# Autodesk Inventor assembly: Robot Assembly
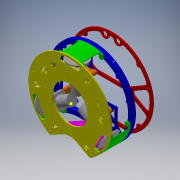
[picture p0: Inventor's stored thumbnail of the model, 180x180]
Saved by Autodesk Inventor 2018 (Build 220112000, 112)
## iProperties
Created: 2018-06-13
Part Number: Robot Assembly
Document SubType Name: Assembly
Designer: matth
Author: matth
## Documents named in this file (8)
- C:\Users\matth\Dropbox\M&A\Robotics-2018\Design and Hardware\Joinmax Parts\Robot Assembly.iam
- C:\Users\matth\Dropbox\M&A\Robotics-2018\Design and Hardware\Joinmax Parts\Base Plate.ipt
- C:\Users\matth\Dropbox\M&A\Robotics-2018\Design and Hardware\Joinmax Parts\Wheel Guard.ipt
- C:\Users\matth\Dropbox\M&A\Robotics-2018\Design and Hardware\Joinmax Parts\Joinmax.ipt
- C:\Users\matth\Dropbox\M&A\Robotics-2018\Design and Hardware\Joinmax Parts\Motor Standoff.ipt
- C:\Users\matth\Dropbox\M&A\Robotics-2018\Design and Hardware\Joinmax Parts\TSSP Ring.ipt
- C:\Users\matth\Dropbox\M&A\Robotics-2018\Design and Hardware\Joinmax Parts\Top Plate.ipt
- C:\Users\matth\Dropbox\M&A\Robotics-2018\Design and Hardware\Joinmax Parts\Capture Zone.ipt
## Components (13 placed, 7 different names)
1. Base Plate:1 — Mate:1, Mate:2, Mate:3, Mate:4, Mate:5, Mate:8, Mate:9, Mate:10, Mate:11, Mate:12, Mate:24
2. Wheel Guard:1 — Mate:1, Mate:2
3. Wheel Guard:2 — Mate:4, Mate:5
4. Wheel Guard:3 — Mate:3, Mate:25
5. Joinmax:1 — Mate:11, Mate:12, Mate:16, Mate:17
6. Joinmax:2 — Mate:9, Mate:10, Mate:13, Mate:14
7. Joinmax:3 — Mate:8, Mate:15
8. Motor Standoff:1 — Mate:16, Mate:17
9. Motor Standoff:2 — Mate:15
10. Motor Standoff:3 — Mate:13, Mate:14
11. Capture Zone:1 — Mate:24
12. TSSP Ring:1 — Mate:25
13. Top Plate:1
## Relationships (17: Mate 17)
- Mate:1: Base Plate:1 ↔ Wheel Guard:1
- Mate:2: Base Plate:1 ↔ Wheel Guard:1
- Mate:3: Base Plate:1 ↔ Wheel Guard:3
- Mate:4: Base Plate:1 ↔ Wheel Guard:2
- Mate:5: Base Plate:1 ↔ Wheel Guard:2
- Mate:8: Base Plate:1 ↔ Joinmax:3
- Mate:9: Base Plate:1 ↔ Joinmax:2
- Mate:10: Base Plate:1 ↔ Joinmax:2
- Mate:11: Base Plate:1 ↔ Joinmax:1
- Mate:12: Base Plate:1 ↔ Joinmax:1
- Mate:13: Joinmax:2 ↔ Motor Standoff:3
- Mate:14: Joinmax:2 ↔ Motor Standoff:3
- Mate:15: Joinmax:3 ↔ Motor Standoff:2
- Mate:16: Joinmax:1 ↔ Motor Standoff:1
- Mate:17: Joinmax:1 ↔ Motor Standoff:1
- Mate:24: Base Plate:1 ↔ Capture Zone:1
- Mate:25: Wheel Guard:3 ↔ TSSP Ring:1
